# Autodesk Inventor assembly: Bumper Assembly V2
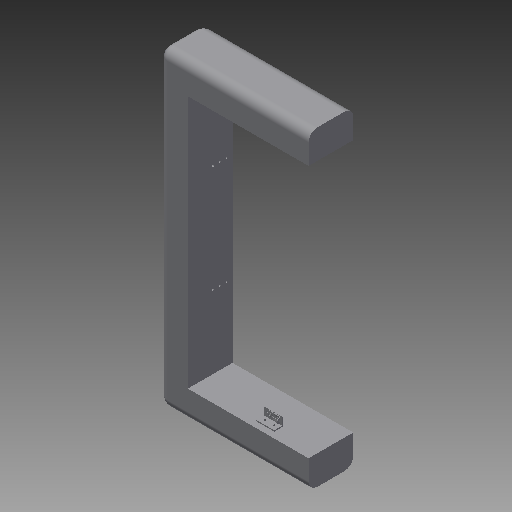
[picture p0: Inventor's stored thumbnail of the model, 512x512]
Saved by Autodesk Inventor 2018 (Build 220112000, 112)
## iProperties
Created: 2020-01-24
Part Number: Bumper Assembly V2
Document SubType Name: Assembly
Designer: S-2512711
Author: S-2512711
## Documents named in this file (4)
- C:\Users\maste\OneDrive\Documents\GitHub\2020CAD\Bumpers\Main Assembly File\Bumper Assembly V2.iam
- C:\Users\maste\OneDrive\Documents\GitHub\2020CAD\Bumpers\Part Files\Bumper Side V2.ipt
- C:\Users\maste\OneDrive\Documents\GitHub\2020CAD\Bumpers\Part Files\Bumper Attachment 1.iam
- C:\Users\maste\OneDrive\Documents\GitHub\2020CAD\Bumpers\Part Files\Bumper Attachment 2.iam
## Components (3 placed, 3 different names)
1. Bumper Side V2:1 — Mate:1, Mate:2, Mate:3, Mate:4, Mate:5, Mate:6
2. Bumper Attachment 1:1 [sub-assembly] — Mate:1, Mate:2, Mate:3
3. Bumper Attachment 2:1 [sub-assembly] — Mate:4, Mate:5, Mate:6
## Relationships (6: Mate 6)
- Mate:1: Bumper Side V2:1 ↔ Bumper Attachment 1:1
- Mate:2: Bumper Side V2:1 ↔ Bumper Attachment 1:1
- Mate:3: Bumper Side V2:1 ↔ Bumper Attachment 1:1
- Mate:4: Bumper Side V2:1 ↔ Bumper Attachment 2:1
- Mate:5: Bumper Side V2:1 ↔ Bumper Attachment 2:1
- Mate:6: Bumper Side V2:1 ↔ Bumper Attachment 2:1
